# Autodesk Inventor assembly: Board
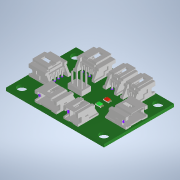
[picture p0: Inventor's stored thumbnail of the model, 180x180]
Saved by Autodesk Inventor 2022 (Build 260153000, 153)
## iProperties
Created: 2024-02-02
Part Number: Board
Document SubType Name: Assembly
Designer: Paul
Author: Paul
## Documents named in this file (8)
- C:\Users\Paul\Documents\Inventor\2024 Mavericks\Swerve\Board\Board.iam
- C:\Users\Paul\Documents\Inventor\2024 Mavericks\Swerve\Board\board.ipt
- C:\Users\Paul\Documents\Inventor\2024 Mavericks\Swerve\Board\Componets\55935-0210_stp\559350210.ipt
- C:\Users\Paul\Documents\Inventor\2024 Mavericks\Swerve\Board\Componets\55935-0410_stp\559350410.ipt
- C:\Users\Paul\Documents\Inventor\2024 Mavericks\Swerve\Board\Male_Pin_1x3.ipt
- C:\Users\Paul\Documents\Inventor\2024 Mavericks\Swerve\Board\Soldering_Jig_Swerve.ipt
- C:\Users\Paul\Documents\Inventor\2024 Mavericks\Swerve\Board\LED 1206 Grn.ipt
- C:\Users\Paul\Documents\Inventor\2024 Mavericks\Swerve\Board\LED 1206 Red.ipt
## Components (13 placed, 7 different names)
1. board:1 — Mate:1, Mate:2, Mate:3, Mate:4, Mate:5, Mate:6, Mate:7, Mate:8, Mate:9, Mate:10, Mate:11, Mate:12, Mate:13, Mate:14, Mate:15, Mate:16, Mate:17, Mate:18, Mate:19, Mate:20, Mate:21, Mate:22, Mate:23, Mate:24, Mate:25, Mate:26, Mate:27, Mate:28, Mate:29, Flush:2, Flush:3, Flush:5
2. 559350210:1 — Mate:17, Mate:20, Mate:21
3. 559350210:2 — Mate:16, Mate:18, Mate:19
4. 559350210:3 — Mate:13, Mate:14, Mate:15
5. 559350410:1 — Mate:7, Mate:8, Mate:9
6. 559350410:2 — Mate:10, Mate:11, Mate:12
7. 559350410:3 — Mate:4, Mate:5, Mate:6, Flush:1
8. 559350410:4 — Mate:1, Mate:2, Mate:3
9. Male_Pin_1x3:1 — Mate:23, Mate:26, Mate:27
10. Male_Pin_1x3:2 — Mate:22, Mate:24, Mate:25
11. Soldering_Jig_Swerve:1 — Flush:1
12. LED 1206 Grn:1 — Mate:28, Flush:2, Flush:4, Flush:5
13. LED 1206 Red:1 — Mate:29, Flush:3, Flush:4
## Relationships (34: Mate 29, Flush 5)
- Mate:1: board:1 ↔ 559350410:4
- Mate:2: board:1 ↔ 559350410:4
- Mate:3: board:1 ↔ 559350410:4
- Mate:4: board:1 ↔ 559350410:3
- Mate:5: board:1 ↔ 559350410:3
- Mate:6: board:1 ↔ 559350410:3
- Mate:7: board:1 ↔ 559350410:1
- Mate:8: board:1 ↔ 559350410:1
- Mate:9: board:1 ↔ 559350410:1
- Mate:10: board:1 ↔ 559350410:2
- Mate:11: board:1 ↔ 559350410:2
- Mate:12: board:1 ↔ 559350410:2
- Mate:13: board:1 ↔ 559350210:3
- Mate:14: board:1 ↔ 559350210:3
- Mate:15: board:1 ↔ 559350210:3
- Mate:16: board:1 ↔ 559350210:2
- Mate:17: board:1 ↔ 559350210:1
- Mate:18: board:1 ↔ 559350210:2
- Mate:19: board:1 ↔ 559350210:2
- Mate:20: board:1 ↔ 559350210:1
- Mate:21: board:1 ↔ 559350210:1
- Mate:22: board:1 ↔ Male_Pin_1x3:2
- Mate:23: board:1 ↔ Male_Pin_1x3:1
- Mate:24: board:1 ↔ Male_Pin_1x3:2
- Mate:25: board:1 ↔ Male_Pin_1x3:2
- Mate:26: board:1 ↔ Male_Pin_1x3:1
- Mate:27: board:1 ↔ Male_Pin_1x3:1
- Flush:1: 559350410:3 ↔ Soldering_Jig_Swerve:1
- Mate:28: board:1 ↔ LED 1206 Grn:1
- Mate:29: board:1 ↔ LED 1206 Red:1
- Flush:2 (16.218 mm): board:1 ↔ LED 1206 Grn:1
- Flush:3 (20.536 mm): board:1 ↔ LED 1206 Red:1
- Flush:4: LED 1206 Grn:1 ↔ LED 1206 Red:1
- Flush:5 (17.958 mm): board:1 ↔ LED 1206 Grn:1
